# Autodesk Inventor assembly: リンク_ふともも_後ろ_1
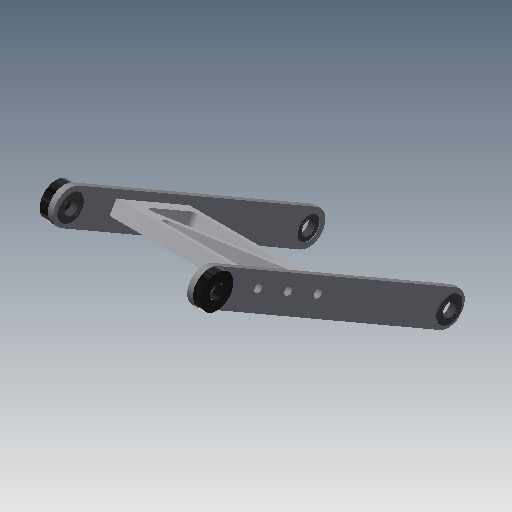
[picture p0: Inventor's stored thumbnail of the model, 512x512]
Saved by Autodesk Inventor 2017.3 (Build 213256000, 256)
## iProperties
Created: 2016-04-27
Part Number: リンク_ふともも_後ろ_1
Document SubType Name: Assembly
Designer: hiroaki
Mass: 38.6491 g
Surface Area: 115.476 cm^2
Volume: 9.14719 cm^3
Density: 4.22524 g/cm^3
Author: hiroaki
## Documents named in this file (6)
- C:\Users\haya\Desktop\GankenKun0_5\下半身\リンク\ふともも\リンク_ふともも_後ろ_1.iam
- C:\Users\haya\Desktop\GankenKun0_5\下半身\リンク\ふともも\リンク_ふともも_メインフレーム_1_2.ipt
- C:\Users\haya\Desktop\GankenKun0_5\既製品\NSK_RB_MF85ZZ\MF85ZZ.iam
- C:\Users\haya\Desktop\GankenKun0_5\下半身\リンク\スペーサ\膝_同軸_スペーサ_1_3.ipt
- C:\Users\haya\Desktop\GankenKun0_5\既製品\CC-0512-30B.ipt
- C:\Users\haya\Desktop\GankenKun0_5\下半身\リンク\ふともも\リンク_ふともも_サブフレーム_1_2(予備案).ipt
## Components (9 placed, 5 different names)
1. リンク_ふともも_メインフレーム_1_2:1 — 挿入:9, 挿入:10, 挿入:19, 挿入:27, 挿入:28, 挿入:29
2. リンク_ふともも_メインフレーム_1_2:2 — 挿入:8, 挿入:17, 挿入:26, 挿入:30, 挿入:31, 挿入:32
3. MF85ZZ:1 [sub-assembly] — 挿入:17
4. MF85ZZ:2 [sub-assembly] — 挿入:8
5. MF85ZZ:3 [sub-assembly] — 挿入:10
6. MF85ZZ:4 [sub-assembly] — 挿入:9
7. 膝_同軸_スペーサ_1_3:1 — 挿入:19
8. CC-0512-30B:1 — 挿入:26
9. リンク_ふともも_サブフレーム_1_2(予備案):1 — 挿入:27, 挿入:28, 挿入:29, 挿入:30, 挿入:31, 挿入:32
## Relationships (12: Insert 12)
- 挿入:8 [Insert]: リンク_ふともも_メインフレーム_1_2:2 ↔ MF85ZZ:2
- 挿入:9 [Insert]: リンク_ふともも_メインフレーム_1_2:1 ↔ MF85ZZ:4
- 挿入:10 [Insert]: リンク_ふともも_メインフレーム_1_2:1 ↔ MF85ZZ:3
- 挿入:17 [Insert]: リンク_ふともも_メインフレーム_1_2:2 ↔ MF85ZZ:1
- 挿入:19 [Insert]: リンク_ふともも_メインフレーム_1_2:1 ↔ 膝_同軸_スペーサ_1_3:1
- 挿入:26 [Insert]: リンク_ふともも_メインフレーム_1_2:2 ↔ CC-0512-30B:1
- 挿入:27 [Insert]: リンク_ふともも_メインフレーム_1_2:1 ↔ リンク_ふともも_サブフレーム_1_2(予備案):1
- 挿入:28 [Insert]: リンク_ふともも_メインフレーム_1_2:1 ↔ リンク_ふともも_サブフレーム_1_2(予備案):1
- 挿入:29 [Insert]: リンク_ふともも_メインフレーム_1_2:1 ↔ リンク_ふともも_サブフレーム_1_2(予備案):1
- 挿入:30 [Insert]: リンク_ふともも_メインフレーム_1_2:2 ↔ リンク_ふともも_サブフレーム_1_2(予備案):1
- 挿入:31 [Insert]: リンク_ふともも_メインフレーム_1_2:2 ↔ リンク_ふともも_サブフレーム_1_2(予備案):1
- 挿入:32 [Insert]: リンク_ふともも_メインフレーム_1_2:2 ↔ リンク_ふともも_サブフレーム_1_2(予備案):1
